# Autodesk Inventor assembly: Assembly1
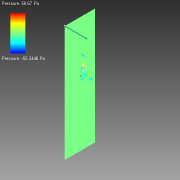
[picture p0: Inventor's stored thumbnail of the model, 180x180]
Saved by Autodesk Inventor 2015 (Build 190159000, 159)
## iProperties
Created: 2015-03-28
Part Number: Assembly1
Document SubType Name: Assembly
Designer: C4f4s
Author: C4f4s
## Documents named in this file (4)
- C:\Users\C4f4s\Desktop\Invictus_2015\Projects\Car\Assembly1.iam
- C:\Users\C4f4s\Desktop\Invictus_2015\Projects\Car\2015 Front Spoiler 1.ipt
- C:\Users\C4f4s\Desktop\Invictus_2015\Projects\Car\2015 Project 5b.ipt
- C:\Users\C4f4s\Desktop\Invictus_2015\Projects\Car\2015 Back Spoiler 1.ipt
## Components (3 placed, 3 different names)
1. 2015 Front Spoiler 1:1 — Flush:1
2. 2015 Project 5b:1 — Flush:1, Flush:2, Mate:1, Flush:3
3. 2015 Back Spoiler 1:1 — Flush:2, Mate:1, Flush:3
## Relationships (4: Flush 3, Mate 1)
- Flush:1: 2015 Front Spoiler 1:1 ↔ 2015 Project 5b:1
- Flush:2 (32 mm): 2015 Project 5b:1 ↔ 2015 Back Spoiler 1:1
- Mate:1: 2015 Project 5b:1 ↔ 2015 Back Spoiler 1:1
- Flush:3 (-21 mm): 2015 Project 5b:1 ↔ 2015 Back Spoiler 1:1
